# Autodesk Inventor assembly: HS 36T Gear, Square_MIR
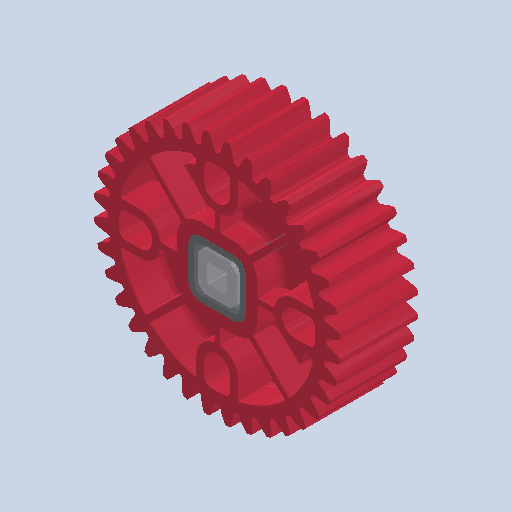
[picture p0: Inventor's stored thumbnail of the model, 512x512]
Saved by Autodesk Inventor 2024 (Build 280153000, 153)
## iProperties
Created: 2022-08-02
Part Number: HS 36T Gear, Square_MIR
Document SubType Name: Assembly
Designer: ismae
Author: ylu12
## Documents named in this file (3)
- C:\Users\ismae\Desktop\VEX\CAD 2023\VEX-CAD-Inventor\Motion\Gears\HS Gear\HS 36T Gear, Square_MIR.iam
- C:\Users\ismae\Desktop\VEX\CAD 2023\VEX-CAD-Inventor\Motion\HS Shaft Adapter Square_MIR.ipt
- C:\Users\ismae\Desktop\VEX\CAD 2023\VEX-CAD-Inventor\Motion\Gears\Reference Files\HS 36T Gear, No Insert_MIR.ipt
## Components (2 placed, 2 different names)
1. HS Shaft Adapter Square_MIR:1 — Nivelación:2, Coincidencia:4, Coincidencia:3
2. HS 36T Gear, No Insert_MIR:1 — Coincidencia:10, Coincidencia:9, Nivelación:5
## Relationships (6: Mate 4, Flush 2)
- Nivelación:2 [Flush] (-6.35 mm): HS Shaft Adapter Square_MIR:1
- Coincidencia:4 [Mate]: HS Shaft Adapter Square_MIR:1
- Coincidencia:3 [Mate]: HS Shaft Adapter Square_MIR:1
- Coincidencia:10 [Mate]: HS 36T Gear, No Insert_MIR:1
- Coincidencia:9 [Mate]: HS 36T Gear, No Insert_MIR:1
- Nivelación:5 [Flush]: HS 36T Gear, No Insert_MIR:1
